# Autodesk Inventor assembly: SE tarjedas de AD DC
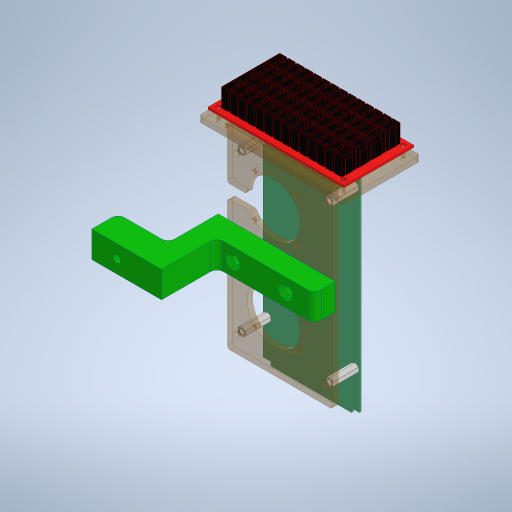
[picture p0: Inventor's stored thumbnail of the model, 512x512]
Saved by Autodesk Inventor 2024.2 (Build 282272000, 272)
## iProperties
Created: 2024-08-27
Part Number: SE tarjedas de AD DC
Document SubType Name: Assembly
Designer: ja.restrepo1
Author: ja.restrepo1
## Documents named in this file (6)
- I:\MICROMECANICA\ALTAS ENERGIAS\Deteccion de Muones\Detectores centelladores\Partes Detector Centellador\SE Tarjetas IC DC\SSE tarjedas de AD DC.iam
- I:\MICROMECANICA\ALTAS ENERGIAS\Deteccion de Muones\Detectores centelladores\Partes Detector Centellador\SE Tarjetas IC DC\Soporte IC KAEN\Conector IC DC.ipt
- I:\MICROMECANICA\ALTAS ENERGIAS\Deteccion de Muones\Detectores centelladores\Partes Detector Centellador\SE Tarjetas IC DC\Soporte IC KAEN\Tarjeta IC DC.ipt
- I:\MICROMECANICA\ALTAS ENERGIAS\Deteccion de Muones\Detectores centelladores\Partes Detector Centellador\SE Tarjetas IC DC\Soporte IC KAEN\Placa soporte TIC DC.ipt
- I:\MICROMECANICA\ALTAS ENERGIAS\Deteccion de Muones\Detectores centelladores\Partes Detector Centellador\SE Tarjetas IC DC\Soporte IC KAEN\Marco conectores IC DC.ipt
- I:\MICROMECANICA\ALTAS ENERGIAS\Deteccion de Muones\Detectores centelladores\Partes Detector Centellador\SE Tarjetas IC DC\Soporte IC KAEN\unión placa soporte TIC DC.ipt
## Components (5 placed, 5 different names)
1. Conector IC DC:1 — Mate:1, Flush:1, Mate:2, Mate:3, Angle:1, Angle:2, Flush:2, Flush:3, Mate:4, Mate:8, Mate:9, Mate:10
2. Tarjeta IC DC:1 — Angle:1, Angle:2, Flush:2, Flush:3, Mate:4, Mate:5, Mate:6, Mate:7
3. Placa soporte TIC DC:1 — Mate:5, Mate:6, Mate:7, Mate:11, Mate:12, Mate:13
4. Marco conectores IC DC:1 — Mate:8, Mate:9, Mate:10
5. unión placa soporte TIC DC:1 — Mate:11, Mate:12, Mate:13
## Relationships (18: Mate 13, Flush 3, Angle 2)
- Mate:1: Conector IC DC:1
- Flush:1: Conector IC DC:1
- Mate:2: Conector IC DC:1
- Mate:3: Conector IC DC:1
- Angle:1 (180 deg): Conector IC DC:1 ↔ Tarjeta IC DC:1
- Angle:2 (0 deg): Conector IC DC:1 ↔ Tarjeta IC DC:1
- Flush:2: Conector IC DC:1 ↔ Tarjeta IC DC:1
- Flush:3 (-1 mm): Conector IC DC:1 ↔ Tarjeta IC DC:1
- Mate:4 (-6.5 mm): Conector IC DC:1 ↔ Tarjeta IC DC:1
- Mate:5: Tarjeta IC DC:1 ↔ Placa soporte TIC DC:1
- Mate:6: Tarjeta IC DC:1 ↔ Placa soporte TIC DC:1
- Mate:7: Tarjeta IC DC:1 ↔ Placa soporte TIC DC:1
- Mate:8: Conector IC DC:1 ↔ Marco conectores IC DC:1
- Mate:9: Conector IC DC:1 ↔ Marco conectores IC DC:1
- Mate:10 (4 mm): Conector IC DC:1 ↔ Marco conectores IC DC:1
- Mate:11: Placa soporte TIC DC:1 ↔ unión placa soporte TIC DC:1
- Mate:12: Placa soporte TIC DC:1 ↔ unión placa soporte TIC DC:1
- Mate:13: Placa soporte TIC DC:1 ↔ unión placa soporte TIC DC:1
